# Autodesk Inventor assembly: 組合1
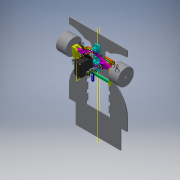
[picture p0: Inventor's stored thumbnail of the model, 180x180]
Saved by Autodesk Inventor 2019 (Build 230136000, 136)
## iProperties
Created: 2020-03-19
Part Number: 組合1
Material: 一般
Document SubType Name: Assembly
Designer: 吳昇峻
Author: 吳昇峻
## Documents named in this file (15)
- C:\Users\user\Desktop\機工實務\0320最終\組合1.iam
- C:\Users\user\Desktop\機工實務\0320最終\a臂鎖.ipt
- C:\Users\user\Desktop\機工實務\0320最終\底盤新.ipt
- C:\Users\user\Desktop\機工實務\0320最終\下a臂.ipt
- C:\Users\user\Desktop\機工實務\0320最終\羊角.ipt
- C:\Users\user\Desktop\機工實務\0320最終\阿克曼長軸.ipt
- C:\Users\user\Desktop\機工實務\0320最終\防傾桿.ipt
- C:\Users\user\Desktop\機工實務\0320最終\轉向軸.ipt
- C:\Users\user\Desktop\機工實務\0320最終\m3_30.ipt
- C:\Users\user\Desktop\機工實務\0320最終\Servomotor.ipt
- C:\Users\user\Desktop\機工實務\0320最終\Servomotor-1.ipt
- C:\Users\user\Desktop\機工實務\0320最終\上底盤新.ipt
- C:\Users\user\Desktop\機工實務\0320最終\前輪.ipt
- C:\Users\user\Desktop\機工實務\0320最終\避震.ipt
- C:\Users\user\Desktop\機工實務\0320最終\避震器上部.ipt
## Components (19 placed, 14 different names)
1. a臂鎖:1 — 貼合:1, 圓柱:1, 圓柱:3, 貼合:3, Cylindrical:18, Mate:16
2. 底盤新:1 — 貼合:1, 圓柱:1, Mate:12, Mate:13, Flush:2
3. 下a臂:2 — 圓柱:3, 貼合:3, 圓柱:4, 貼合:4, Cylindrical:21, Mate:18
4. 羊角:2 — 圓柱:4, 貼合:4, 圓柱:7, Cylindrical:16, Mate:14, Cylindrical:25
5. 羊角:3 — 圓柱:6, 貼合:6, Cylindrical:17, Mate:15, Cylindrical:19, Cylindrical:24, Mate:19, 貼合:20
6. 阿克曼長軸:1 — 圓柱:6, 貼合:6, 圓柱:7, 圓柱:10, 齊平:1, Mate:9
7. 轉向軸:1 — Tangent:1, Cylindrical:15, Mate:9, Mate:10, Mate:11
8. m3_30:1 — 圓柱:10, 齊平:1, Tangent:1
9. Servomotor:1 — Cylindrical:14, Mate:8
10. Servomotor-1:1 — Cylindrical:14, Mate:8, Cylindrical:15, Mate:10, Mate:11
11. 上底盤新:1 — Mate:12, Mate:13, Flush:2
12. 前輪:1 — Cylindrical:16, Mate:14
13. 前輪:2 — Cylindrical:17, Mate:15
14. 下a臂:3 — Cylindrical:18, Mate:16, Cylindrical:19, Cylindrical:20, Mate:17, 貼合:20
15. 避震:1 — Cylindrical:20, Mate:17, Cylindrical:22
16. 避震:2 — Cylindrical:21, Mate:18, Cylindrical:23
17. 避震器上部:1 — Cylindrical:22
18. 避震器上部:2 — Cylindrical:23
19. 防傾桿:1 — Cylindrical:24, Cylindrical:25, Mate:19
## Relationships (38: CylindricalJoint 18, Mate 17, Flush 2, Tangent 1)
- 貼合:1 [Mate]: a臂鎖:1 ↔ 底盤新:1
- 圓柱:1 [CylindricalJoint]: a臂鎖:1 ↔ 底盤新:1
- 圓柱:3 [CylindricalJoint]: a臂鎖:1 ↔ 下a臂:2
- 貼合:3 [Mate] (1 mm): a臂鎖:1 ↔ 下a臂:2
- 圓柱:4 [CylindricalJoint]: 下a臂:2 ↔ 羊角:2
- 貼合:4 [Mate] (0.5 mm): 下a臂:2 ↔ 羊角:2
- 圓柱:6 [CylindricalJoint]: 羊角:3 ↔ 阿克曼長軸:1
- 貼合:6 [Mate] (2 mm): 羊角:3 ↔ 阿克曼長軸:1
- 圓柱:7 [CylindricalJoint]: 羊角:2 ↔ 阿克曼長軸:1
- 圓柱:10 [CylindricalJoint]: 阿克曼長軸:1 ↔ m3_30:1
- 齊平:1 [Flush] (-5 mm): 阿克曼長軸:1 ↔ m3_30:1
- Cylindrical:14: Servomotor:1 ↔ Servomotor-1:1
- Mate:8 (1 mm): Servomotor:1 ↔ Servomotor-1:1
- Tangent:1 (0.3 mm): 轉向軸:1 ↔ m3_30:1
- Cylindrical:15: 轉向軸:1 ↔ Servomotor-1:1
- Mate:9 (3 mm): 阿克曼長軸:1 ↔ 轉向軸:1
- Mate:10: 轉向軸:1 ↔ Servomotor-1:1
- Mate:11: 轉向軸:1 ↔ Servomotor-1:1
- Mate:12: 底盤新:1 ↔ 上底盤新:1
- Mate:13 (35.967 mm): 底盤新:1 ↔ 上底盤新:1
- Flush:2: 底盤新:1 ↔ 上底盤新:1
- Cylindrical:16: 羊角:2 ↔ 前輪:1
- Mate:14 (1 mm): 羊角:2 ↔ 前輪:1
- Cylindrical:17: 羊角:3 ↔ 前輪:2
- Mate:15 (1 mm): 羊角:3 ↔ 前輪:2
- Cylindrical:18: a臂鎖:1 ↔ 下a臂:3
- Mate:16 (1 mm): a臂鎖:1 ↔ 下a臂:3
- Cylindrical:19: 羊角:3 ↔ 下a臂:3
- Cylindrical:20: 下a臂:3 ↔ 避震:1
- Mate:17 (0.3 mm): 下a臂:3 ↔ 避震:1
- Cylindrical:21: 下a臂:2 ↔ 避震:2
- Mate:18 (0.3 mm): 下a臂:2 ↔ 避震:2
- Cylindrical:22: 避震:1 ↔ 避震器上部:1
- Cylindrical:23: 避震:2 ↔ 避震器上部:2
- Cylindrical:24: 羊角:3 ↔ 防傾桿:1
- Cylindrical:25: 羊角:2 ↔ 防傾桿:1
- Mate:19 (1 mm): 羊角:3 ↔ 防傾桿:1
- 貼合:20 [Mate]: 羊角:3 ↔ 下a臂:3
